# Autodesk Inventor assembly: joint4
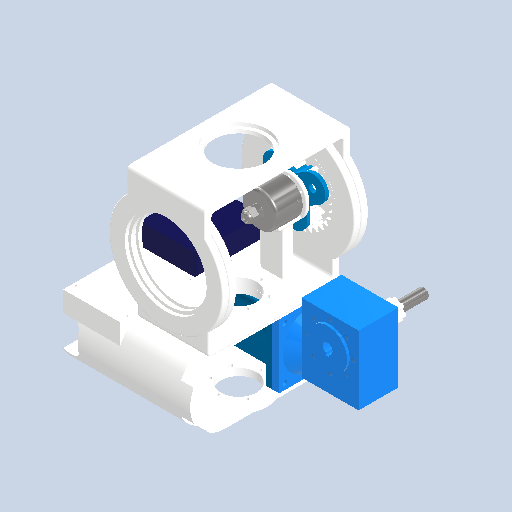
[picture p0: Inventor's stored thumbnail of the model, 512x512]
Saved by Autodesk Inventor 2025.3 (Build 293356030, 356C)
## iProperties
Created: 2025-08-31
Part Number: joint4
Document SubType Name: Assembly
Designer: MSI
Mass: 6375.56 g
Surface Area: 6651.28 cm^2
Volume: 3553.43 cm^3
Density: 1.7942 g/cm^3
Author: MSI
## Documents named in this file (12)
- C:\Users\MSI\Desktop\Project\11. 로봇팔\Robot Arm Model\Robot_Arm_6_v1\joint2.iam
- C:\Users\MSI\Desktop\Project\11. 로봇팔\Robot Arm Model\Robot_Arm_6_v1\motor_holder_1.ipt
- C:\Users\MSI\Desktop\Project\11. 로봇팔\Robot Arm Model\Robot_Arm_6_v1\NMRV30_motor.iam
- C:\Users\MSI\Desktop\Project\11. 로봇팔\Robot Arm Model\Robot_Arm_6_v1\base.ipt
- C:\Users\MSI\Desktop\Project\11. 로봇팔\Robot Arm Model\Robot_Arm_6_v1\frame.ipt
- C:\Users\MSI\Desktop\Project\11. 로봇팔\Robot Arm Model\Robot_Arm_6_v1\encoder.ipt
- C:\Users\MSI\Desktop\Project\11. 로봇팔\Robot Arm Model\Robot_Arm_6_v1\belt_pulley_1.ipt
- C:\Users\MSI\Desktop\Project\11. 로봇팔\Robot Arm Model\Robot_Arm_6_v1\belt_pulley_2.ipt
- C:\Users\MSI\Desktop\Project\11. 로봇팔\Robot Arm Model\Robot_Arm_6_v1\motor_shaft.ipt
- C:\Users\MSI\Desktop\Project\11. 로봇팔\Robot Arm Model\Robot_Arm_6_v1\motor_driver.ipt
- C:\Users\MSI\Desktop\Project\11. 로봇팔\Robot Arm Model\Robot_Arm_6_v1\joint3_meteor.iam
- C:\Users\MSI\Desktop\Project\11. 로봇팔\Robot Arm Model\Robot_Arm_6_v1\encoder_frame.ipt
## Components (11 placed, 11 different names)
1. base:1 — 회전:1, 강체:5, 강체:15
2. frame:1 — 회전:1, 강체:8, 강체:13
3. encoder:1 — 강체:14
4. NMRV30_motor:1 [sub-assembly] — 강체:3, 강체:9, 강체:11
5. motor_holder_1:1 — 강체:3, 강체:5, 강체:12
6. 동기식 풀리1:2 — 강체:9
7. 동기식 풀리2:2 — 강체:8
8. motor_shaft:1 — 강체:11
9. motor_driver:2 — 강체:12
10. joint3_meteor:1 [sub-assembly] — 강체:13
11. encoder_frame:1 — 강체:14, 강체:15
## Relationships (10: WeldJoint 9, RevoluteJoint 1)
- 회전:1 [RevoluteJoint]: base:1 ↔ frame:1
- 강체:3 [WeldJoint]: NMRV30_motor:1 ↔ motor_holder_1:1
- 강체:5 [WeldJoint]: base:1 ↔ motor_holder_1:1
- 강체:8 [WeldJoint]: frame:1 ↔ 동기식 풀리2:2
- 강체:9 [WeldJoint] (9 mm): NMRV30_motor:1 ↔ 동기식 풀리1:2
- 강체:11 [WeldJoint]: NMRV30_motor:1 ↔ motor_shaft:1
- 강체:12 [WeldJoint]: motor_holder_1:1 ↔ motor_driver:2
- 강체:13 [WeldJoint]: frame:1 ↔ joint3_meteor:1
- 강체:14 [WeldJoint]: encoder:1 ↔ encoder_frame:1
- 강체:15 [WeldJoint]: base:1 ↔ encoder_frame:1
